# Autodesk Inventor assembly: Assembly_Lasergroup_wPickup_v1
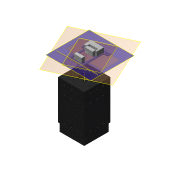
[picture p0: Inventor's stored thumbnail of the model, 180x180]
Saved by Autodesk Inventor 2019 (Build 230136000, 136)
## iProperties
Created: 2019-04-21
Part Number: Assembly_Lasergroup_wPickup_v1
Document SubType Name: Assembly
Designer: diederichbenedict
Author: diederichbenedict
## Documents named in this file (3)
- C:\Users\diederichbenedict\Dropbox\Dokumente\Promotion\PROJECTS\STORMoChip\INVENTOR\Nanoscopy-on-a-cheap\Assembly_Lasergroup_wPickup_v1.iam
- C:\Users\diederichbenedict\Dropbox\Dokumente\Promotion\PROJECTS\STORMoChip\INVENTOR\Nanoscopy-on-a-cheap\00_LASER_640nm.ipt
- C:\Users\diederichbenedict\Dropbox\Dokumente\Promotion\PROJECTS\STORMoChip\INVENTOR\Nanoscopy-on-a-cheap\00_KES400.iam
## Components (2 placed, 2 different names)
1. 00_LASER_640nm:1 — Mate:2, Angle:1, Mate:3
2. 00_KES400:1 [sub-assembly] — Mate:2, Angle:1, Mate:3
## Relationships (3: Mate 2, Angle 1)
- Mate:2: 00_LASER_640nm:1 ↔ 00_KES400:1
- Angle:1 (0 deg): 00_LASER_640nm:1 ↔ 00_KES400:1
- Mate:3 (20 mm): 00_LASER_640nm:1 ↔ 00_KES400:1
